# Autodesk Inventor assembly: Blade Assembly
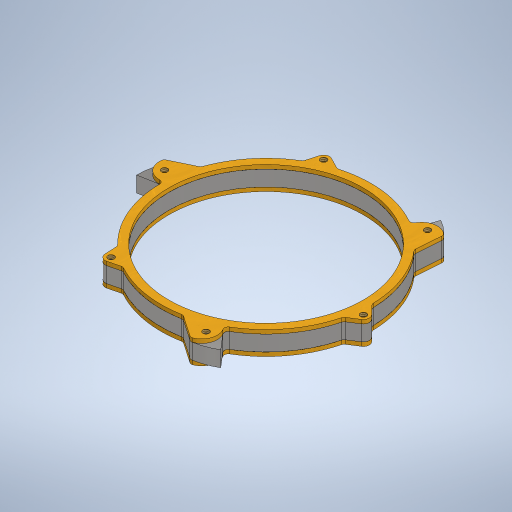
[picture p0: Inventor's stored thumbnail of the model, 512x512]
Saved by Autodesk Inventor 2023.2 (Build 272271000, 271)
## iProperties
Created: 2023-06-25
Part Number: Blade Assembly
Document SubType Name: Assembly
Designer: Nathan Cai
Mass: 717.373 g
Surface Area: 513.949 cm^2
Volume: 87.8971 cm^3
Density: 8.16151 g/cm^3
Author: Nathan Cai
## Documents named in this file (3)
- E:\Documents\Inventor\Moon Cake V1.01\Blade Assembly.iam
- E:\Documents\Inventor\Moon Cake V1.01\Blade.ipt
- E:\Documents\Inventor\Moon Cake V1.01\Blade - Bushing.ipt
## Components (3 placed, 2 different names)
1. Blade:1 — Mate:1, Mate:2, Mate:3, Mate:4, Mate:5, Mate:6
2. Blade - Bushing:1 — Mate:1, Mate:3, Mate:6
3. Blade - Bushing:2 — Mate:2, Mate:4, Mate:5
## Relationships (6: Mate 6)
- Mate:1: Blade:1 ↔ Blade - Bushing:1
- Mate:2: Blade:1 ↔ Blade - Bushing:2
- Mate:3: Blade:1 ↔ Blade - Bushing:1
- Mate:4: Blade:1 ↔ Blade - Bushing:2
- Mate:5: Blade:1 ↔ Blade - Bushing:2
- Mate:6: Blade:1 ↔ Blade - Bushing:1
